# Autodesk Inventor assembly: DoorAssembly
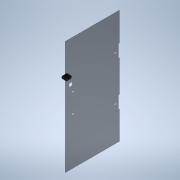
[picture p0: Inventor's stored thumbnail of the model, 180x180]
Saved by Autodesk Inventor 2021 (Build 250183000, 183)
## iProperties
Created: 2021-05-13
Part Number: DoorAssembly
Document SubType Name: Assembly
Designer: gisen
Author: gisen
## Documents named in this file (3)
- D:\GitProjects\CAD-Data\CuboidAccessories\SecurityBox\Assemblies\DoorAssembly.iam
- D:\GitProjects\CAD-Data\CuboidAccessories\SecurityBox\3DPrintedParts\DoorLockHook.ipt
- D:\GitProjects\CAD-Data\CuboidAccessories\SecurityBox\Plates\DoorPlate.ipt
## Components (2 placed, 2 different names)
1. DoorLockHook:1 — メイト:1, メイト:5, メイト:6
2. DoorPlate:1 — メイト:1, メイト:2, メイト:3, メイト:4, メイト:5, メイト:6
## Relationships (6: Mate 6)
- メイト:1 [Mate]: DoorLockHook:1 ↔ DoorPlate:1
- メイト:2 [Mate]: DoorPlate:1
- メイト:3 [Mate]: DoorPlate:1
- メイト:4 [Mate]: DoorPlate:1
- メイト:5 [Mate]: DoorLockHook:1 ↔ DoorPlate:1
- メイト:6 [Mate]: DoorLockHook:1 ↔ DoorPlate:1
